# Autodesk Inventor assembly: Assembly
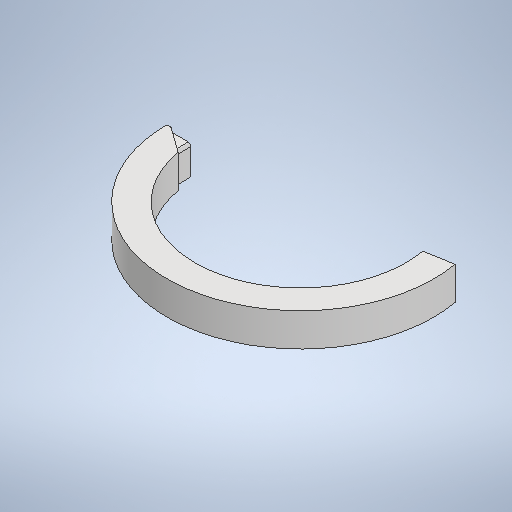
[picture p0: Inventor's stored thumbnail of the model, 512x512]
Saved by Autodesk Inventor 2025 (Build 290162000, 162)
## iProperties
Created: 2026-01-08
Part Number: Assembly
Document SubType Name: Assembly
Designer: tapen
Author: tapen
## Documents named in this file (3)
- C:\Users\tapen\OneDrive\Desktop\Vesna Milosevic-Zdjelar\InertiaKit\Assembly.iam
- C:\Users\tapen\OneDrive\Desktop\Vesna Milosevic-Zdjelar\InertiaKit\InertiaKitOuter.ipt
- C:\Users\tapen\OneDrive\Desktop\Vesna Milosevic-Zdjelar\InertiaKit\InertiaKitInner.ipt
## Components (2 placed, 2 different names)
1. InertiaKitOuter:1 — Mate:1, Flush:1, Flush:2
2. InertiaKitInner:1 — Mate:1, Flush:1, Flush:2
## Relationships (3: Flush 2, Mate 1)
- Mate:1: InertiaKitOuter:1 ↔ InertiaKitInner:1
- Flush:1: InertiaKitOuter:1 ↔ InertiaKitInner:1
- Flush:2: InertiaKitOuter:1 ↔ InertiaKitInner:1
